# Autodesk Inventor assembly: arm-third2
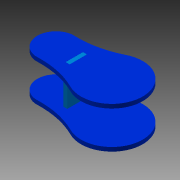
[picture p0: Inventor's stored thumbnail of the model, 180x180]
Saved by Autodesk Inventor 2013 (Build 170138000, 138)
## iProperties
Created: 2012-09-09
Part Number: arm-third2
Document SubType Name: Assembly
Designer: frankenteddy
Author: frankenteddy
## Documents named in this file (3)
- C:\Users\frankenteddy\Desktop\oshawatt1\arm-third.iam
- C:\Users\frankenteddy\Desktop\oshawatt1\arm-third-front.ipt
- C:\Users\frankenteddy\Desktop\oshawatt1\arm-third-strut.ipt
## Components (3 placed, 2 different names)
1. arm-third-front:1 — Mate:4, Mate:5, Mate:6
2. arm-third-strut:1 — Mate:1, Mate:2, Mate:3, Mate:4, Mate:5, Mate:6
3. arm-third-front:2 — Mate:1, Mate:2, Mate:3
## Relationships (6: Mate 6)
- Mate:1: arm-third-strut:1 ↔ arm-third-front:2
- Mate:2: arm-third-strut:1 ↔ arm-third-front:2
- Mate:3: arm-third-strut:1 ↔ arm-third-front:2
- Mate:4: arm-third-front:1 ↔ arm-third-strut:1
- Mate:5: arm-third-front:1 ↔ arm-third-strut:1
- Mate:6: arm-third-front:1 ↔ arm-third-strut:1
